# Autodesk Inventor assembly: TractioniPod
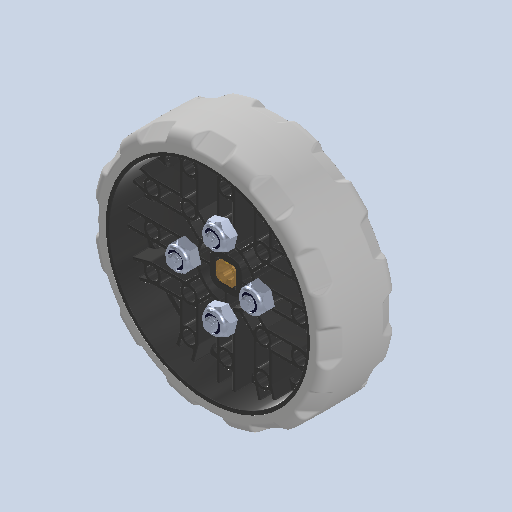
[picture p0: Inventor's stored thumbnail of the model, 512x512]
Saved by Autodesk Inventor 2025.1 (Build 291241020, 241B)
## iProperties
Created: 2024-10-26
Part Number: TractioniPod
Document SubType Name: Assembly
Designer: Juan
Author: Juan
## Documents named in this file (9)
- C:\Users\Hunter Mathis\Documents\GitHub\ATUM-V5RC-High-Stakes-CAD\Robot\Subassemblies\TractioniPod.iam
- C:\Users\Hunter Mathis\Documents\GitHub\ATUM-V5RC-High-Stakes-CAD\VEX-CAD-Inventor\Motion\Gears\HS Gear\HS 48T Gear, Circle.iam
- C:\Users\Juan\Documents\GitHub\ATUM-VRC-High-Stakes-CAD\VEX-CAD-Inventor\Motion\Gears\HS Gear.iam
- C:\Users\Hunter Mathis\Documents\GitHub\ATUM-V5RC-High-Stakes-CAD\VEX-CAD-Inventor\Structure\Hardware\Screw Steel - Star\SScrew Star Threaded 1.250.ipt
- C:\Users\Juan\Documents\GitHub\ATUM-VRC-High-Stakes-CAD\VEX-CAD-Inventor\Structure\Hardware\Screw Steel - Star.ipt
- C:\Users\Hunter Mathis\Documents\GitHub\ATUM-V5RC-High-Stakes-CAD\VEX-CAD-Inventor\Structure\Hardware\Nut Thin Nylock.ipt
- C:\Users\Hunter Mathis\Documents\GitHub\ATUM-V5RC-High-Stakes-CAD\VEX-CAD-Inventor\Motion\HS Shaft Adapter Circle.ipt
- C:\Users\Hunter Mathis\Documents\GitHub\ATUM-V5RC-High-Stakes-CAD\VEX-CAD-Inventor\Motion\Wheels\Traction Wheel\3.25 Traction AS, No Insert.iam
- C:\Users\Juan\Documents\GitHub\ATUM-VRC-High-Stakes-CAD\VEX-CAD-Inventor\Motion\Wheels\Traction Wheel.iam
## Components (11 placed, 5 different names)
1. 3.25 Traction AS, No Insert:1 [sub-assembly] — Mate:13, Mate:14, Mate:15, Mate:16, Mate:17, Mate:18, Mate:19, Flush:1
2. HS 48T Gear, Circle:1 [sub-assembly] — Mate:6, Mate:7, Mate:13, Mate:14, Mate:15, Mate:16, Mate:17
3. HS Shaft Adapter Circle:1 — Mate:18, Mate:19, Flush:1
4. SScrew Star Threaded 1.250:1 — Mate:6, Mate:7, Mate:8
5. Nut Thin Nylock:1 — Mate:8
6. SScrew Star Threaded 1.250:2
7. Nut Thin Nylock:2
8. SScrew Star Threaded 1.250:3
9. Nut Thin Nylock:3
10. SScrew Star Threaded 1.250:4
11. Nut Thin Nylock:4
## Component patterns: (4 elements, first: SScrew Star Threaded 1.250:1 + Nut Thin Nylock:1)
## Relationships (11: Mate 10, Flush 1)
- Mate:6: HS 48T Gear, Circle:1 ↔ SScrew Star Threaded 1.250:1
- Mate:7: HS 48T Gear, Circle:1 ↔ SScrew Star Threaded 1.250:1
- Mate:8: SScrew Star Threaded 1.250:1 ↔ Nut Thin Nylock:1
- Mate:13: 3.25 Traction AS, No Insert:1 ↔ HS 48T Gear, Circle:1
- Mate:14: 3.25 Traction AS, No Insert:1 ↔ HS 48T Gear, Circle:1
- Mate:15: 3.25 Traction AS, No Insert:1 ↔ HS 48T Gear, Circle:1
- Mate:16: 3.25 Traction AS, No Insert:1 ↔ HS 48T Gear, Circle:1
- Mate:17: 3.25 Traction AS, No Insert:1 ↔ HS 48T Gear, Circle:1
- Mate:18: 3.25 Traction AS, No Insert:1 ↔ HS Shaft Adapter Circle:1
- Mate:19: 3.25 Traction AS, No Insert:1 ↔ HS Shaft Adapter Circle:1
- Flush:1: 3.25 Traction AS, No Insert:1 ↔ HS Shaft Adapter Circle:1
